# Autodesk Inventor assembly: castor
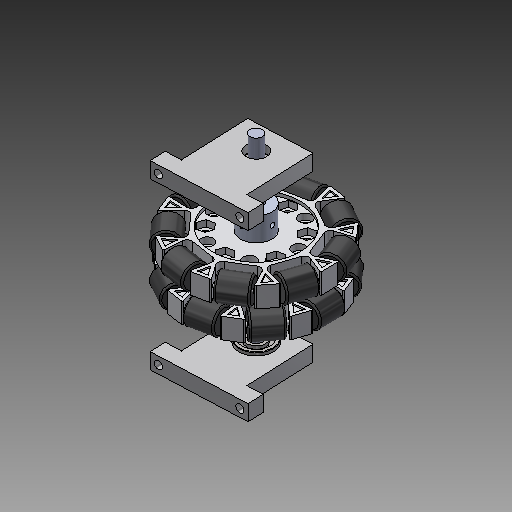
[picture p0: Inventor's stored thumbnail of the model, 512x512]
Saved by Autodesk Inventor 2018 (Build 220112000, 112)
## iProperties
Created: 2017-05-04
Part Number: castor
Document SubType Name: Assembly
Designer: AYUSH SHUKLA
Author: AYUSH SHUKLA
## Documents named in this file (6)
- C:\Study\BTP2\Robomuse Inventor CAD\Caster\caster.iam
- C:\Study\BTP2\Robomuse Inventor CAD\Caster\caster_shaft.ipt
- C:\Study\BTP2\Robomuse Inventor CAD\Caster\caster_bearing.ipt
- C:\Study\BTP2\Robomuse Inventor CAD\Caster\radial ball bearing_68_iso_ISO 15 RBB - 108 - 8,SI,NC,8_68.ipt
- C:\Study\BTP2\Robomuse Inventor CAD\Caster\final_wheel.iam
- C:\Study\BTP2\Robomuse Inventor CAD\Caster\axle.ipt
## Components (8 placed, 5 different names)
1. caster_shaft:1
2. caster_bearing:1 — Flush:2, Mate:14
3. radial ball bearing_68_iso_ISO 15 RBB - 108 - 8,SI,NC,8_68:1
4. caster_bearing:2 — Flush:2
5. radial ball bearing_68_iso_ISO 15 RBB - 108 - 8,SI,NC,8_68:2
6. final_wheel:1 [sub-assembly]
7. final_wheel:2 [sub-assembly] — Mate:14
8. axle:1
## Relationships (16: Mate 14, Flush 2)
- [Mate]: caster_bearing:1 ↔ radial ball bearing_68_iso_ISO 15 RBB - 108 - 8,SI,NC,8_68:1
- [Mate]: caster_bearing:1 ↔ radial ball bearing_68_iso_ISO 15 RBB - 108 - 8,SI,NC,8_68:1
- [Mate]: caster_shaft:1 ↔ radial ball bearing_68_iso_ISO 15 RBB - 108 - 8,SI,NC,8_68:1
- [Mate]: caster_bearing:2 ↔ radial ball bearing_68_iso_ISO 15 RBB - 108 - 8,SI,NC,8_68:2
- [Mate]: caster_bearing:2 ↔ radial ball bearing_68_iso_ISO 15 RBB - 108 - 8,SI,NC,8_68:2
- [Mate]: caster_shaft:1 ↔ caster_bearing:2
- [Flush] (-9.8 mm): caster_shaft:1 ↔ caster_bearing:2
- [Mate]: final_wheel:1 ↔ final_wheel:2
- [Mate]: final_wheel:1 ↔ final_wheel:2
- [Mate] (10 mm): final_wheel:1 ↔ final_wheel:2
- [Mate]: final_wheel:2 ↔ axle:1
- [Mate]: final_wheel:2 ↔ axle:1
- [Mate]: caster_shaft:1 ↔ axle:1
- [Mate] (33.7 mm): caster_bearing:2 ↔ final_wheel:1
- Flush:2: caster_bearing:1 ↔ caster_bearing:2
- Mate:14 (33.7 mm): caster_bearing:1 ↔ final_wheel:2
## Named parameters: d52_d49 = 0 mm, d53_d50 = 0 mm
